# Autodesk Inventor assembly: ChainTensioner_Assembly_v2
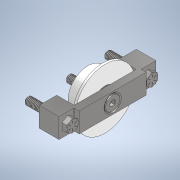
[picture p0: Inventor's stored thumbnail of the model, 180x180]
Saved by Autodesk Inventor 2022 (Build 260153000, 153)
## iProperties
Created: 2021-06-19
Part Number: ChainTensioner_Assembly_v2
Document SubType Name: Assembly
Designer: M3rob
Author: M3rob
## Documents named in this file (7)
- C:\Users\M3rob\Documents\GrabCAD\FireBird 250 Pound Gaming Machine\Drafts\FrameDrafts\Draft_04\Assemblies\Final Draft 04 Assemblies\ChainTensioner_Assembly_v2.iam
- C:\Users\M3rob\Documents\GrabCAD\FireBird 250 Pound Gaming Machine\Drafts\FrameDrafts\Draft_04\Weapon System\Chain_Tensioner\ChainTensioner_v2.ipt
- C:\Users\M3rob\Documents\GrabCAD\FireBird 250 Pound Gaming Machine\Drafts\FrameDrafts\Draft_04\Hardware\60355K601_ChainTensioner_Bearing.ipt
- C:\Users\M3rob\Documents\GrabCAD\FireBird 250 Pound Gaming Machine\Drafts\FrameDrafts\Draft_04\Hardware\91259A714_ChainTensioner_ShoulderScrew.ipt
- C:\Users\M3rob\Documents\GrabCAD\FireBird 250 Pound Gaming Machine\Drafts\FrameDrafts\Draft_04\Weapon System\Chain_Tensioner\UHMW_Idler.ipt
- C:\Users\M3rob\Documents\GrabCAD\FireBird 250 Pound Gaming Machine\Drafts\FrameDrafts\Draft_04\Hardware\ChainTensionerBearingShim.ipt
- C:\Users\M3rob\Documents\GrabCAD\FireBird 250 Pound Gaming Machine\Drafts\FrameDrafts\Draft_04\Hardware\91257A632_LongChassisScrew.ipt
## Components (9 placed, 6 different names)
1. ChainTensioner_v2:1 — Mate:11, Mate:12, Mate:13, Mate:14, Mate:15, Angle:1, Mate:16, Angle:2, Mate:17
2. 60355K601_ChainTensioner_Bearing:1
3. 91259A714_ChainTensioner_ShoulderScrew:1 — Mate:11, Mate:12
4. 60355K601_ChainTensioner_Bearing:2
5. UHMW_Idler:1
6. ChainTensionerBearingShim:1
7. ChainTensionerBearingShim:2 — Mate:13
8. 91257A632_LongChassisScrew:1 — Mate:14, Mate:15, Angle:1
9. 91257A632_LongChassisScrew:2 — Mate:16, Angle:2, Mate:17
## Relationships (19: Mate 17, Angle 2)
- [Mate]: 60355K601_ChainTensioner_Bearing:1 ↔ 91259A714_ChainTensioner_ShoulderScrew:1
- [Mate]: 91259A714_ChainTensioner_ShoulderScrew:1 ↔ 60355K601_ChainTensioner_Bearing:2
- [Mate]: 60355K601_ChainTensioner_Bearing:2 ↔ UHMW_Idler:1
- [Mate]: 60355K601_ChainTensioner_Bearing:2 ↔ UHMW_Idler:1
- [Mate]: 60355K601_ChainTensioner_Bearing:1 ↔ UHMW_Idler:1
- [Mate]: 60355K601_ChainTensioner_Bearing:1 ↔ UHMW_Idler:1
- [Mate]: 91259A714_ChainTensioner_ShoulderScrew:1 ↔ ChainTensionerBearingShim:2
- [Mate]: 60355K601_ChainTensioner_Bearing:2 ↔ ChainTensionerBearingShim:1
- [Mate]: 91259A714_ChainTensioner_ShoulderScrew:1 ↔ ChainTensionerBearingShim:1
- [Mate]: 60355K601_ChainTensioner_Bearing:1 ↔ ChainTensionerBearingShim:2
- Mate:11: ChainTensioner_v2:1 ↔ 91259A714_ChainTensioner_ShoulderScrew:1
- Mate:12: ChainTensioner_v2:1 ↔ 91259A714_ChainTensioner_ShoulderScrew:1
- Mate:13: ChainTensioner_v2:1 ↔ ChainTensionerBearingShim:2
- Mate:14: ChainTensioner_v2:1 ↔ 91257A632_LongChassisScrew:1
- Mate:15: ChainTensioner_v2:1 ↔ 91257A632_LongChassisScrew:1
- Angle:1 (0 deg): ChainTensioner_v2:1 ↔ 91257A632_LongChassisScrew:1
- Mate:16: ChainTensioner_v2:1 ↔ 91257A632_LongChassisScrew:2
- Angle:2 (0 deg): ChainTensioner_v2:1 ↔ 91257A632_LongChassisScrew:2
- Mate:17: ChainTensioner_v2:1 ↔ 91257A632_LongChassisScrew:2
